# Autodesk Inventor assembly: Joshuas Mistakes
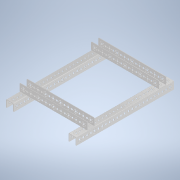
[picture p0: Inventor's stored thumbnail of the model, 180x180]
Saved by Autodesk Inventor 2020.1 (Build 241239000, 239)
## iProperties
Created: 2019-09-10
Part Number: Joshuas Mistakes
Document SubType Name: Assembly
Designer: alphaomega
Author: alphaomega
## Documents named in this file (3)
- C:\Users\alphaomega\Documents\Joshuas Mistakes.iam
- C:\Users\alphaomega\Documents\GitHub\AO_Robotics\CAD\Parts Kits\FTC Tetrix KOP Organized (7-24-19)\Frame Hardware\Tetrix_39069.ipt
- C:\Users\alphaomega\Documents\GitHub\AO_Robotics\CAD\Parts Kits\FTC Tetrix KOP Organized (7-24-19)\Frame Hardware\Tetrix_39068.ipt
## Components (4 placed, 2 different names)
1. Tetrix_39069:1 — Rigid:2, Rotational:1, Flush:1
2. Tetrix_39068:1 — Rigid:2
3. Tetrix_39069:2
4. Tetrix_39068:2 — Rotational:1, Flush:1
## Relationships (3: WeldJoint 1, RevoluteJoint 1, Flush 1)
- Rigid:2 [WeldJoint]: Tetrix_39069:1 ↔ Tetrix_39068:1
- Rotational:1 [RevoluteJoint]: Tetrix_39069:1 ↔ Tetrix_39068:2
- Flush:1: Tetrix_39069:1 ↔ Tetrix_39068:2
